# Autodesk Inventor assembly: Right Leg NEO
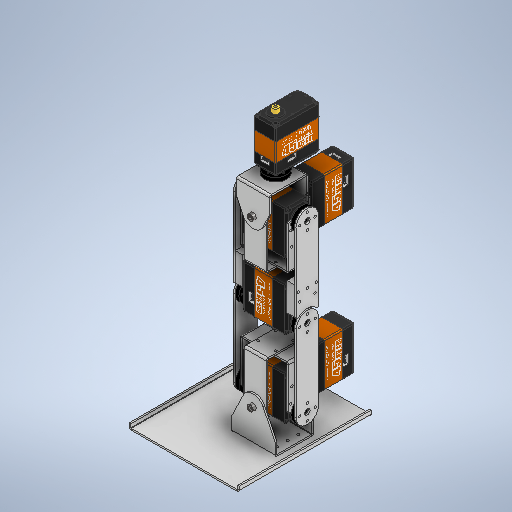
[picture p0: Inventor's stored thumbnail of the model, 512x512]
Saved by Autodesk Inventor 2025.2 (Build 292293000, 293)
## iProperties
Created: 2025-07-04
Part Number: Right Leg NEO
Document SubType Name: Assembly
Designer: User
Author: User
## Documents named in this file (18)
- C:\Users\User\Documents\The Maverick's Files\College 3-3\로보인 프로젝트\RHp_Humanoid_ver1\Assembly\Right Leg NEO.iam
- C:\Users\User\Documents\The Maverick's Files\College 3-3\로보인 프로젝트\RHp_Humanoid_ver1\Part\HTD-45H, Horn\HTD-45H\HTD-45H.ipt
- C:\Users\User\Documents\The Maverick's Files\College 3-3\로보인 프로젝트\RHp_Humanoid_ver1\Part\HTD-45H, Horn\Horn\Bottom Horn.ipt
- C:\Users\User\Documents\The Maverick's Files\College 3-3\로보인 프로젝트\RHp_Humanoid_ver1\Part\HTD-45H, Horn\Horn\Top Horn.ipt
- C:\Users\User\Documents\The Maverick's Files\College 3-3\로보인 프로젝트\RHp_Humanoid_ver1\Part\Frame\Leg\axis_7_top_frame.ipt
- C:\Users\User\Documents\The Maverick's Files\College 3-3\로보인 프로젝트\RHp_Humanoid_ver1\Part\Frame\Leg\axis_9_bottom_frame.ipt
- C:\Users\User\Documents\The Maverick's Files\College 3-3\로보인 프로젝트\RHp_Humanoid_ver1\Part\Frame\Leg\axis_8_bottom_frame.ipt
- C:\Users\User\Documents\The Maverick's Files\College 3-3\로보인 프로젝트\RHp_Humanoid_ver1\Part\Frame\Leg\axis_8_10_connector_frame.ipt
- C:\Users\User\Documents\The Maverick's Files\College 3-3\로보인 프로젝트\RHp_Humanoid_ver1\Part\Frame\Leg\3D_printed_part.ipt
- C:\Users\User\Documents\The Maverick's Files\College 3-3\로보인 프로젝트\RHp_Humanoid_ver1\Part\Frame\Leg\axis_10_11-connector_frame.ipt
- C:\Users\User\Documents\The Maverick's Files\College 3-3\로보인 프로젝트\RHp_Humanoid_ver1\Part\Frame\Leg\axis_11_top_frame.ipt
- C:\Users\User\Documents\The Maverick's Files\College 3-3\로보인 프로젝트\RHp_Humanoid_ver1\Part\Frame\Leg\axis_12_top_frame.ipt
- C:\Users\User\Documents\The Maverick's Files\College 3-3\로보인 프로젝트\RHp_Humanoid_ver1\Part\Frame\Leg\axis_12_bottom_frame(top).ipt
- C:\Users\User\Documents\The Maverick's Files\College 3-3\로보인 프로젝트\RHp_Humanoid_ver1\Part\Frame\Leg\axis_12_bottom_frame(bottom).ipt
- C:\Users\User\Documents\The Maverick's Files\College 3-3\로보인 프로젝트\RHp_Humanoid_ver1\Part\Bolt, Bearing, Nut, Washer\M3x8.ipt
- C:\Users\User\Documents\The Maverick's Files\College 3-3\로보인 프로젝트\RHp_Humanoid_ver1\Part\Bolt, Bearing, Nut, Washer\M3 Nut.ipt
- C:\Users\User\Documents\The Maverick's Files\College 3-3\로보인 프로젝트\RHp_Humanoid_ver1\Part\Bolt, Bearing, Nut, Washer\M3 Washer.ipt
- C:\Users\User\Documents\The Maverick's Files\College 3-3\로보인 프로젝트\RHp_Humanoid_ver1\Part\Frame\Leg\3D_printed_part_2.ipt
## Components (34 placed, 17 different names)
1. HTD-45H:1 — Flush:2, Rotational:1, Flush:5, Mate:12
2. HTD-45H:2 — Rotational:2, Mate:4, Mate:5, Flush:4
3. HTD-45H:3 — Mate:9, Mate:10, Mate:11, Rotational:3, Rotational:4
4. HTD-45H:4 — Flush:14, Flush:15, Mate:13, Mate:14, Rotational:5, Rotational:6, Flush:27, Flush:30
5. HTD-45H:5 — Mate:17, Mate:18, Mate:19, Rotational:13, Rotational:14
6. HTD-45H:6 — Rotational:9, Mate:21, Mate:23, Flush:22
7. Bottom Horn:1 — Rotational:1, Mate:1, Mate:2, Mate:3
8. Bottom Horn:2 — Rotational:4, Rigid:5
9. Bottom Horn:3 — Rotational:5, Rigid:8
10. Bottom Horn:4 — Rotational:13, Rigid:18
11. Top Horn:1 — Rotational:2, Rigid:4
12. Top Horn:2 — Rotational:3, Rigid:6
13. Top Horn:3 — Rotational:6, Rigid:7
14. Top Horn:4 — Rotational:14, Rigid:19
15. Top Horn:5 — Rotational:9, Rigid:16
16. axis_9_bottom_frame:1 — Mate:4, Mate:5, Flush:4, Mate:6, Mate:7, Mate:8, Rigid:13
17. axis_8_bottom_frame:1 — Mate:6, Mate:7, Mate:8, Mate:9, Mate:10, Mate:11
18. axis_8_10_connector_frame:1 — Rigid:6, Flush:14, Flush:15, Mate:14, Mate:16, Flush:28
19. axis_8_10_connector_frame:2 — Rigid:5, Mate:13, Mate:25, Flush:29
20. 3D_printed_part:2 — Mate:16, Flush:27, Flush:28
21. axis_10_11-connector_frame:1 — Rigid:7, Rigid:19
22. axis_10_11-connector_frame:2 — Rigid:8, Rigid:18
23. axis_11_top_frame:1 — Mate:17, Mate:18, Mate:19, Mate:20, Flush:20, Flush:21
24. axis_12_top_frame:1 — Mate:20, Flush:20, Flush:21, Mate:21, Mate:23, Flush:22, Rigid:15, Rigid:17
25. axis_12_bottom_frame(top):1 — Mate:24, Flush:23, Flush:24, Rotational:12, Rigid:16
26. axis_7_top_frame:1 — Mate:1, Mate:2, Mate:3, Rigid:4, Rigid:12, Rotational:10
27. axis_12_bottom_frame(bottom):1 — Mate:24, Flush:23, Flush:24
28. M3x8:1 — Rotational:10
29. M3 Nut:1 — Rigid:15
30. M3 Nut:2 — Rigid:13
31. M3 Washer:1 — Rigid:17
32. M3 Washer:2 — Rigid:12
33. M3x8:2 — Rotational:12
34. 3D_printed_part_2:1 — Mate:25, Flush:29, Flush:30
## Relationships (60: Mate 23, Flush 14, WeldJoint 12, RevoluteJoint 11)
- Flush:2: HTD-45H:1
- Rotational:1 [RevoluteJoint]: HTD-45H:1 ↔ Bottom Horn:1
- Mate:1: Bottom Horn:1 ↔ axis_7_top_frame:1
- Mate:2: Bottom Horn:1 ↔ axis_7_top_frame:1
- Mate:3 (-14.43 mm): Bottom Horn:1 ↔ axis_7_top_frame:1
- Rotational:2 [RevoluteJoint]: HTD-45H:2 ↔ Top Horn:1
- Rigid:4 [WeldJoint]: Top Horn:1 ↔ axis_7_top_frame:1
- Mate:4: HTD-45H:2 ↔ axis_9_bottom_frame:1
- Mate:5: HTD-45H:2 ↔ axis_9_bottom_frame:1
- Flush:4 (-11.5 mm): HTD-45H:2 ↔ axis_9_bottom_frame:1
- Mate:6: axis_9_bottom_frame:1 ↔ axis_8_bottom_frame:1
- Mate:7: axis_9_bottom_frame:1 ↔ axis_8_bottom_frame:1
- Mate:8 (1.5 mm): axis_9_bottom_frame:1 ↔ axis_8_bottom_frame:1
- Mate:9: HTD-45H:3 ↔ axis_8_bottom_frame:1
- Mate:10: HTD-45H:3 ↔ axis_8_bottom_frame:1
- Mate:11 (8.5 mm): HTD-45H:3 ↔ axis_8_bottom_frame:1
- Flush:5: HTD-45H:1
- Mate:12: HTD-45H:1
- Rotational:3 [RevoluteJoint]: HTD-45H:3 ↔ Top Horn:2
- Rotational:4 [RevoluteJoint]: HTD-45H:3 ↔ Bottom Horn:2
- Rigid:5 [WeldJoint]: Bottom Horn:2 ↔ axis_8_10_connector_frame:2
- Rigid:6 [WeldJoint]: Top Horn:2 ↔ axis_8_10_connector_frame:1
- Flush:14: HTD-45H:4 ↔ axis_8_10_connector_frame:1
- Flush:15 (-7.07 mm): HTD-45H:4 ↔ axis_8_10_connector_frame:1
- Mate:13: HTD-45H:4 ↔ axis_8_10_connector_frame:2
- Mate:14 (-30.1 mm): HTD-45H:4 ↔ axis_8_10_connector_frame:1
- Mate:16: axis_8_10_connector_frame:1 ↔ 3D_printed_part:2
- Rotational:5 [RevoluteJoint]: HTD-45H:4 ↔ Bottom Horn:3
- Rotational:6 [RevoluteJoint]: HTD-45H:4 ↔ Top Horn:3
- Rigid:7 [WeldJoint]: Top Horn:3 ↔ axis_10_11-connector_frame:1
- Rigid:8 [WeldJoint]: Bottom Horn:3 ↔ axis_10_11-connector_frame:2
- Mate:17: HTD-45H:5 ↔ axis_11_top_frame:1
- Mate:18 (8.5 mm): HTD-45H:5 ↔ axis_11_top_frame:1
- Mate:19: HTD-45H:5 ↔ axis_11_top_frame:1
- Mate:20: axis_11_top_frame:1 ↔ axis_12_top_frame:1
- Flush:20: axis_11_top_frame:1 ↔ axis_12_top_frame:1
- Flush:21 (8.5 mm): axis_11_top_frame:1 ↔ axis_12_top_frame:1
- Rotational:9 [RevoluteJoint]: HTD-45H:6 ↔ Top Horn:5
- Mate:21: HTD-45H:6 ↔ axis_12_top_frame:1
- Mate:23: HTD-45H:6 ↔ axis_12_top_frame:1
- Flush:22 (11.5 mm): HTD-45H:6 ↔ axis_12_top_frame:1
- Mate:24: axis_12_bottom_frame(top):1 ↔ axis_12_bottom_frame(bottom):1
- Flush:23: axis_12_bottom_frame(top):1 ↔ axis_12_bottom_frame(bottom):1
- Flush:24 (20 mm): axis_12_bottom_frame(top):1 ↔ axis_12_bottom_frame(bottom):1
- Rigid:12 [WeldJoint]: axis_7_top_frame:1 ↔ M3 Washer:2
- Rotational:10 [RevoluteJoint]: axis_7_top_frame:1 ↔ M3x8:1
- Rigid:13 [WeldJoint]: axis_9_bottom_frame:1 ↔ M3 Nut:2
- Rotational:12 [RevoluteJoint]: axis_12_bottom_frame(top):1 ↔ M3x8:2
- Rigid:15 [WeldJoint]: axis_12_top_frame:1 ↔ M3 Nut:1
- Rigid:16 [WeldJoint]: Top Horn:5 ↔ axis_12_bottom_frame(top):1
- Flush:27 (4 mm): HTD-45H:4 ↔ 3D_printed_part:2
- Flush:28: axis_8_10_connector_frame:1 ↔ 3D_printed_part:2
- Rigid:17 [WeldJoint]: axis_12_top_frame:1 ↔ M3 Washer:1
- Rotational:13 [RevoluteJoint]: HTD-45H:5 ↔ Bottom Horn:4
- Rigid:18 [WeldJoint]: Bottom Horn:4 ↔ axis_10_11-connector_frame:2
- Rotational:14 [RevoluteJoint]: HTD-45H:5 ↔ Top Horn:4
- Rigid:19 [WeldJoint]: Top Horn:4 ↔ axis_10_11-connector_frame:1
- Mate:25: axis_8_10_connector_frame:2 ↔ 3D_printed_part_2:1
- Flush:29: axis_8_10_connector_frame:2 ↔ 3D_printed_part_2:1
- Flush:30 (4 mm): HTD-45H:4 ↔ 3D_printed_part_2:1
